# Autodesk Inventor assembly: PILLARSCELLCASE21700ASSEMBLY
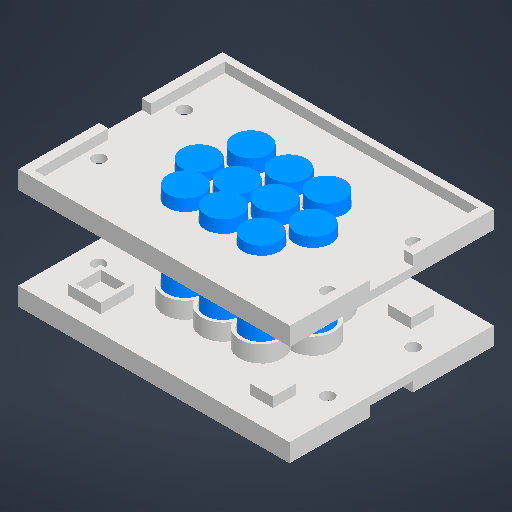
[picture p0: Inventor's stored thumbnail of the model, 512x512]
Saved by Autodesk Inventor 2025.2 (Build 292293000, 293)
## iProperties
Created: 2025-03-05
Part Number: PILLARSCELLCASE21700ASSEMBLY
Document SubType Name: Assembly
Designer: cbast
Author: cbast
## Documents named in this file (3)
- C:\Users\cbast\OneDrive\Documents\GitHub\Smart-Pack-for-Advanced-Research-and-Control\variations\Camden\V0.2\PILLARSCELLCASE21700ASSEMBLY.iam
- C:\Users\cbast\OneDrive\Documents\GitHub\Smart-Pack-for-Advanced-Research-and-Control\variations\Camden\V0.1\21700(Blue).ipt
- C:\Users\cbast\OneDrive\Documents\GitHub\Smart-Pack-for-Advanced-Research-and-Control\variations\Camden\V0.2\PILLARSCELLCASE21700.ipt
## Components (12 placed, 2 different names)
1. 21700(Blue):1 — Mate:2
2. 21700(Blue):2 — Mate:4
3. 21700(Blue):3 — Mate:1
4. 21700(Blue):4 — Mate:5
5. 21700(Blue):5 — Mate:3
6. 21700(Blue):6 — Mate:6
7. 21700(Blue):7 — Mate:7
8. 21700(Blue):8 — Mate:10
9. 21700(Blue):9 — Mate:9
10. 21700(Blue):10 — Mate:8
11. PILLARSCELLCASE21700:1 — Flush:1, Flush:2, Mate:1, Mate:2, Mate:3, Mate:4, Mate:5, Mate:6, Mate:7, Mate:8, Mate:9, Mate:10
12. PILLARSCELLCASE21700:2 — Flush:1, Flush:2
## Relationships (12: Mate 10, Flush 2)
- Flush:1: PILLARSCELLCASE21700:1 ↔ PILLARSCELLCASE21700:2
- Flush:2: PILLARSCELLCASE21700:1 ↔ PILLARSCELLCASE21700:2
- Mate:1: 21700(Blue):3 ↔ PILLARSCELLCASE21700:1
- Mate:2: 21700(Blue):1 ↔ PILLARSCELLCASE21700:1
- Mate:3: 21700(Blue):5 ↔ PILLARSCELLCASE21700:1
- Mate:4: 21700(Blue):2 ↔ PILLARSCELLCASE21700:1
- Mate:5: 21700(Blue):4 ↔ PILLARSCELLCASE21700:1
- Mate:6: 21700(Blue):6 ↔ PILLARSCELLCASE21700:1
- Mate:7: 21700(Blue):7 ↔ PILLARSCELLCASE21700:1
- Mate:8: 21700(Blue):10 ↔ PILLARSCELLCASE21700:1
- Mate:9: 21700(Blue):9 ↔ PILLARSCELLCASE21700:1
- Mate:10: 21700(Blue):8 ↔ PILLARSCELLCASE21700:1
